# Autodesk Inventor assembly: Side
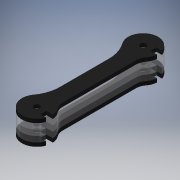
[picture p0: Inventor's stored thumbnail of the model, 180x180]
Saved by Autodesk Inventor 2017 (Build 210142000, 142)
## iProperties
Created: 2017-04-18
Part Number: Side
Document SubType Name: Assembly
Designer: jeffkub
Author: jeffkub
## Documents named in this file (3)
- C:\Projects\nixie-clock\mechanical\Side.iam
- C:\Projects\nixie-clock\mechanical\Spacer1.ipt
- C:\Projects\nixie-clock\mechanical\Spacer2.ipt
## Components (5 placed, 2 different names)
1. Spacer1:1 — Flush:1, Flush:2, Flush:3, Mate:1
2. Spacer2:1 — Flush:4, Flush:5, Mate:1, Mate:2
3. Spacer2:2 — Flush:6, Flush:7, Mate:2, Mate:3
4. Spacer2:3 — Flush:8, Flush:9, Mate:3, Mate:4
5. Spacer1:2 — Flush:10, Flush:11, Mate:4
## Relationships (15: Flush 11, Mate 4)
- Flush:1: Spacer1:1
- Flush:2: Spacer1:1
- Flush:3: Spacer1:1
- Flush:4: Spacer2:1
- Flush:5: Spacer2:1
- Flush:6: Spacer2:2
- Flush:7: Spacer2:2
- Flush:8: Spacer2:3
- Flush:9: Spacer2:3
- Flush:10: Spacer1:2
- Flush:11: Spacer1:2
- Mate:1: Spacer1:1 ↔ Spacer2:1
- Mate:2: Spacer2:1 ↔ Spacer2:2
- Mate:3: Spacer2:2 ↔ Spacer2:3
- Mate:4: Spacer2:3 ↔ Spacer1:2
